# Autodesk Inventor assembly: сборка_балансирного_вала
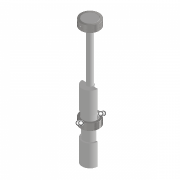
[picture p0: Inventor's stored thumbnail of the model, 180x180]
Saved by Autodesk Inventor 2021 (Build 250183000, 183)
## iProperties
Created: 2021-06-15
Part Number: сборка_балансирного_вала
Document SubType Name: Assembly
Designer: panda
Mass: 337.794 g
Surface Area: 525.747 cm^2
Volume: 184.106 cm^3
Density: 1.83477 g/cm^3
Author: panda
## Documents named in this file (3)
- C:\Users\panda\Desktop\vkrb\сборка\сборка_балансирного_вала.iam
- C:\Users\panda\Desktop\vkrb\сборка\балансирный_вал.ipt
- C:\Users\panda\Documents\Inventor\Content Center Files\R2021\ru-RU\Bearing 24000 GOST 4657-82\Подшипники 4024906 ГОСТ 4657-82.ipt
## Components (3 placed, 2 different names)
1. балансирный_вал:1 — Совмещение:2, Совмещение:3, Совмещение:4, Совмещение:5, Совмещение:6, Совмещение:7, Совмещение:8
2. Подшипники 24000 ГОСТ 4657-82 4024906:3 — Совмещение:2, Совмещение:7
3. Подшипники 24000 ГОСТ 4657-82 4024906:4 — Совмещение:3, Совмещение:8
## Relationships (7: Mate 7)
- Совмещение:2 [Mate]: балансирный_вал:1 ↔ Подшипники 24000 ГОСТ 4657-82 4024906:3
- Совмещение:3 [Mate]: балансирный_вал:1 ↔ Подшипники 24000 ГОСТ 4657-82 4024906:4
- Совмещение:4 [Mate]: балансирный_вал:1
- Совмещение:5 [Mate]: балансирный_вал:1
- Совмещение:6 [Mate]: балансирный_вал:1
- Совмещение:7 [Mate]: балансирный_вал:1 ↔ Подшипники 24000 ГОСТ 4657-82 4024906:3
- Совмещение:8 [Mate]: балансирный_вал:1 ↔ Подшипники 24000 ГОСТ 4657-82 4024906:4
